# Autodesk Inventor assembly: levels
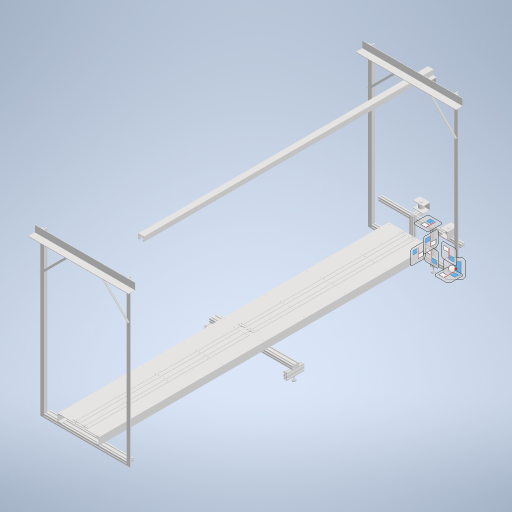
[picture p0: Inventor's stored thumbnail of the model, 512x512]
Saved by Autodesk Inventor 2023 (Build 270158030, 158C)
## iProperties
Created: 2023-02-18
Part Number: levels
Document SubType Name: Assembly
Designer: jeremyy
Author: jeremyy
## Documents named in this file (4)
- \\andrew.ad.cmu.edu\users\users1\jeremyy\Documents\Inventor\CMU Bridge\New folder\levels.iam
- \\andrew.ad.cmu.edu\users\users1\jeremyy\Documents\Inventor\CMU Bridge\New folder\Section 1.iam
- \\andrew.ad.cmu.edu\users\users1\jeremyy\Documents\Inventor\CMU Bridge\New folder\LongStrut84Sec1.ipt
- \\andrew.ad.cmu.edu\users\users1\jeremyy\Documents\Inventor\CMU Bridge\New folder\Gear.iam
## Components (3 placed, 3 different names)
1. Section 1:1 [sub-assembly] — Mate:1, Mate:2, Flush:1
2. LongStrut84Sec1:1 — Mate:1, Mate:2, Flush:1, Mate:3, Flush:2, Flush:3
3. Gear:1 [sub-assembly] — Mate:3, Flush:2, Flush:3
## Relationships (6: Mate 3, Flush 3)
- Mate:1: Section 1:1 ↔ LongStrut84Sec1:1
- Mate:2 (279.4 mm): Section 1:1 ↔ LongStrut84Sec1:1
- Flush:1 (-127 mm): Section 1:1 ↔ LongStrut84Sec1:1
- Mate:3: LongStrut84Sec1:1 ↔ Gear:1
- Flush:2: LongStrut84Sec1:1 ↔ Gear:1
- Flush:3 (-12.7 mm): LongStrut84Sec1:1 ↔ Gear:1
